# Autodesk Inventor assembly: openmv_h7
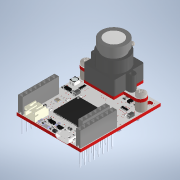
[picture p0: Inventor's stored thumbnail of the model, 180x180]
Saved by Autodesk Inventor 2020 (Build 240168000, 168)
## iProperties
Created: 2019-09-24
Part Number: openmv_h7
Description: STEP AP214
Document SubType Name: Assembly
Designer: 4s
Sending System: SolidWorks 2016
Preprocessor: SwSTEP 2.0
Title: openmv4_h7.STEP
Revision Number: ANY
## Documents named in this file (6)
- C:\Users\4s\Documents\Inventor models\Asterisk\robot_v2\openmv\openmv_h7.iam
- C:\Users\4s\Documents\Inventor models\Asterisk\robot_v2\openmv\openmv4_h7_base_® ã¬®«ç ­¨î.iam
- C:\Users\4s\Documents\Inventor models\Asterisk\robot_v2\openmv\openmv4_ov7725_® ã¬®«ç ­¨î.iam
- C:\Users\4s\Documents\Inventor models\Asterisk\robot_v2\openmv\pan head cross recess screw_iso_ISO 7045 - M2.5 x 5 - Z - 5N.ipt
- C:\Users\4s\Documents\Inventor models\Asterisk\robot_v2\openmv\LENS_Standard_® ã¬®«ç ­¨î.ipt
- C:\Users\4s\Documents\Inventor models\Asterisk\robot_v2\openmv\pan head cross recess screw_iso_ISO 7045 - M1 x 4 - Z - 4S.ipt
## Components (6 placed, 6 different names)
1. openmv4_h7_base_® ã¬®«ç ­¨î_1 [sub-assembly] — Совмещение:4, Совмещение:5, Совмещение:7
2. openmv4_ov7725_® ã¬®«ç ­¨î_2 [sub-assembly] — Совмещение:1, Совмещение:2, Совмещение:3, Совмещение:6, Совмещение:7, Совмещение:8, Совмещение:9
3. pan head cross recess screw_iso_ISO 7045 - M2.5 x 5 - Z - 5N_3 — Совмещение:3, Совмещение:4, Совмещение:9
4. pan head cross recess screw_iso_ISO 7045 - M2.5 x 5 - Z - 5N_4 — Совмещение:5, Совмещение:6, Совмещение:8
5. LENS_Standard_® ã¬®«ç ­¨î_6 — Совмещение:1, Совмещение:2
6. pan head cross recess screw_iso_ISO 7045 - M1 x 4 - Z - 4S_9
## Relationships (9: Mate 9)
- Совмещение:1 [Mate]: openmv4_ov7725_® ã¬®«ç ­¨î_2 ↔ LENS_Standard_® ã¬®«ç ­¨î_6
- Совмещение:2 [Mate] (2 mm): openmv4_ov7725_® ã¬®«ç ­¨î_2 ↔ LENS_Standard_® ã¬®«ç ­¨î_6
- Совмещение:3 [Mate]: openmv4_ov7725_® ã¬®«ç ­¨î_2 ↔ pan head cross recess screw_iso_ISO 7045 - M2.5 x 5 - Z - 5N_3
- Совмещение:4 [Mate]: openmv4_h7_base_® ã¬®«ç ­¨î_1 ↔ pan head cross recess screw_iso_ISO 7045 - M2.5 x 5 - Z - 5N_3
- Совмещение:5 [Mate]: openmv4_h7_base_® ã¬®«ç ­¨î_1 ↔ pan head cross recess screw_iso_ISO 7045 - M2.5 x 5 - Z - 5N_4
- Совмещение:6 [Mate]: openmv4_ov7725_® ã¬®«ç ­¨î_2 ↔ pan head cross recess screw_iso_ISO 7045 - M2.5 x 5 - Z - 5N_4
- Совмещение:7 [Mate]: openmv4_h7_base_® ã¬®«ç ­¨î_1 ↔ openmv4_ov7725_® ã¬®«ç ­¨î_2
- Совмещение:8 [Mate]: openmv4_ov7725_® ã¬®«ç ­¨î_2 ↔ pan head cross recess screw_iso_ISO 7045 - M2.5 x 5 - Z - 5N_4
- Совмещение:9 [Mate]: openmv4_ov7725_® ã¬®«ç ­¨î_2 ↔ pan head cross recess screw_iso_ISO 7045 - M2.5 x 5 - Z - 5N_3
